# Autodesk Inventor assembly: am-0597
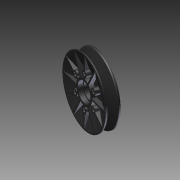
[picture p0: Inventor's stored thumbnail of the model, 180x180]
Saved by Autodesk Inventor 2014 (Build 180170000, 170)
## iProperties
Category: Miscellaneous
Company: Autodesk Inc.
Created: 2013-12-24
Part Number: am-0597
Document SubType Name: Assembly
Designer: Autodesk Inc.
Catalog Web Link: http://www.andymark.com/product-p/am-0592.htm
Vendor: AndyMark
Author: Autodesk Inc.
## Documents named in this file (2)
- D:\Data Folder\FIRST 2014\KOP Parts\Miscellaneous\MISC_Pulley_am-0592.iam
- D:\Data Folder\FIRST 2014\KOP Parts\Miscellaneous\Parts\Misc_Pulley_am-0592.ipt
## Components (2 placed, 1 different names)
1. Misc_Pulley_am-0592:2 — Insert:1, Mate:1
2. Misc_Pulley_am-0592:3 — Insert:1, Mate:1
## Relationships (2: Insert 1, Mate 1)
- Insert:1: Misc_Pulley_am-0592:2 ↔ Misc_Pulley_am-0592:3
- Mate:1: Misc_Pulley_am-0592:2 ↔ Misc_Pulley_am-0592:3
